# Autodesk Inventor assembly: Holder
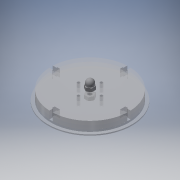
[picture p0: Inventor's stored thumbnail of the model, 180x180]
Saved by Autodesk Inventor 2016 (Build 200138000, 138)
## iProperties
Created: 2018-05-15
Part Number: Holder
Document SubType Name: Assembly
Designer: Phil Erle
Author: Phil Erle
## Documents named in this file (6)
- C:\Users\Phil Erle\Desktop\Adrastea\Holder.iam
- C:\Users\Phil Erle\Desktop\Adrastea\Seconday_End_Bottom.ipt
- C:\Users\Phil Erle\Desktop\Adrastea\Normteile\Muttern\mutter_din934_m6-6.ipt
- C:\Users\Phil Erle\Desktop\Adrastea\Normteile\Muttern\din1587-m6x1ricu3.ipt
- C:\Users\Phil Erle\Desktop\Adrastea\PlexiHalter1.ipt
- C:\Users\Phil Erle\Desktop\Adrastea\PlexiHalter2.ipt
## Components (5 placed, 5 different names)
1. Seconday_End_Bottom:1 — Flush:1, Flush:2, Flush:3, Mate:1, Mate:2, Mate:6, Mate:7, Mate:11
2. mutter_din934_m6-6:1 — Mate:6, Mate:7, Mate:8
3. din1587-m6x1ricu3:1 — Mate:9, Mate:10
4. PlexiHalter1:1 — Mate:1, Mate:3, Mate:4, Mate:5, Mate:8, Mate:11
5. PlexiHalter2:1 — Mate:2, Mate:3, Mate:4, Mate:5, Mate:9, Mate:10
## Relationships (14: Mate 11, Flush 3)
- Flush:1: Seconday_End_Bottom:1
- Flush:2: Seconday_End_Bottom:1
- Flush:3: Seconday_End_Bottom:1
- Mate:1: Seconday_End_Bottom:1 ↔ PlexiHalter1:1
- Mate:2: Seconday_End_Bottom:1 ↔ PlexiHalter2:1
- Mate:3: PlexiHalter1:1 ↔ PlexiHalter2:1
- Mate:4: PlexiHalter1:1 ↔ PlexiHalter2:1
- Mate:5: PlexiHalter1:1 ↔ PlexiHalter2:1
- Mate:6: Seconday_End_Bottom:1 ↔ mutter_din934_m6-6:1
- Mate:7: Seconday_End_Bottom:1 ↔ mutter_din934_m6-6:1
- Mate:8: mutter_din934_m6-6:1 ↔ PlexiHalter1:1
- Mate:9: din1587-m6x1ricu3:1 ↔ PlexiHalter2:1
- Mate:10: din1587-m6x1ricu3:1 ↔ PlexiHalter2:1
- Mate:11: Seconday_End_Bottom:1 ↔ PlexiHalter1:1
